# Autodesk Inventor assembly: Lever Arm
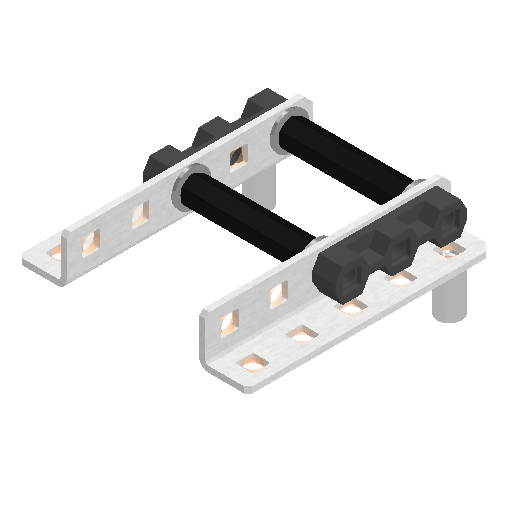
[picture p0: Inventor's stored thumbnail of the model, 512x512]
Saved by Autodesk Inventor 2025 (Build 290162000, 162)
## iProperties
Created: 2025-02-13
Part Number: Lever Arm
Document SubType Name: Assembly
Designer: Averey Ku
Author: Averey Ku
## Documents named in this file (8)
- D:\VEX\High Stakes\CAD\V5\Clamp\Lever Arm.iam
- D:\VEX\High Stakes\CAD\ROBOPROS-CAD-Inventor\Structure\Standoff Rounded\Standoff Rounded.50.ipt
- D:\VEX\High Stakes\CAD\ROBOPROS-CAD-Inventor\Structure\Angle\Aluminum 1x1\Alu Angle 1x1x5.ipt
- D:\VEX\High Stakes\CAD\ROBOPROS-CAD-Inventor\Structure\Standoff\Standoff 1.25.ipt
- D:\VEX\High Stakes\CAD\ROBOPROS-CAD-Inventor\Motion\Spacers\Washer Steel\SWasher .375 OD x .031250.ipt
- D:\VEX\High Stakes\CAD\ROBOPROS-CAD-Inventor\Motion\Spacers\Washer Steel.ipt
- D:\VEX\High Stakes\CAD\ROBOPROS-CAD-Inventor\Motion\Spacers\Washer Steel\SWasher .375 OD x .062500.ipt
- D:\VEX\High Stakes\CAD\ROBOPROS-CAD-Inventor\Motion\Shaft LS\Bearing Flat Low Profile.ipt
## Components (12 placed, 6 different names)
1. Standoff Rounded.50:1
2. Alu Angle 1x1x5:1 — Mate:6, Mate:7
3. Alu Angle 1x1x5:2 — Mate:8
4. Standoff Rounded.50:2
5. Standoff 1.25:1
6. SWasher .375 OD x .031250:1
7. SWasher .375 OD x .062500:2
8. Standoff 1.25:2
9. SWasher .375 OD x .031250:3
10. SWasher .375 OD x .062500:4
11. Bearing Flat Low Profile:1
12. Bearing Flat Low Profile:2
## Relationships (18: Insert 10, Mate 8)
- [Insert]: Standoff Rounded.50:1 ↔ Alu Angle 1x1x5:1
- [Mate]: Alu Angle 1x1x5:1 ↔ Alu Angle 1x1x5:2
- [Insert]: Alu Angle 1x1x5:2 ↔ Standoff Rounded.50:2
- [Insert]: Standoff 1.25:1 ↔ SWasher .375 OD x .062500:2
- [Insert]: Standoff 1.25:1 ↔ SWasher .375 OD x .031250:1
- [Insert]: Alu Angle 1x1x5:2 ↔ SWasher .375 OD x .031250:1
- [Insert]: Standoff 1.25:2 ↔ SWasher .375 OD x .062500:4
- [Insert]: Standoff 1.25:2 ↔ SWasher .375 OD x .031250:3
- [Insert]: Alu Angle 1x1x5:2 ↔ SWasher .375 OD x .031250:3
- [Insert]: Alu Angle 1x1x5:1 ↔ Bearing Flat Low Profile:2
- [Mate]: Alu Angle 1x1x5:1 ↔ Bearing Flat Low Profile:2
- [Insert]: Alu Angle 1x1x5:2 ↔ Bearing Flat Low Profile:1
- [Mate]: Alu Angle 1x1x5:2 ↔ Bearing Flat Low Profile:1
- [Mate]: Alu Angle 1x1x5:1 ↔ SWasher .375 OD x .062500:2
- [Mate] (0.0601 mm): Alu Angle 1x1x5:1 ↔ SWasher .375 OD x .062500:4
- Mate:6: Alu Angle 1x1x5:1
- Mate:7 (17.0957 mm): Alu Angle 1x1x5:1
- Mate:8 (-31.75 mm): Alu Angle 1x1x5:2
## Named parameters: d186_d183 = 0 mm, d187_d184 = 0 mm
